# Autodesk Inventor assembly: keyboard-mockup_cherrymx
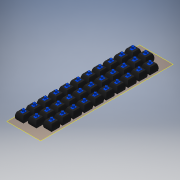
[picture p0: Inventor's stored thumbnail of the model, 180x180]
Saved by Autodesk Inventor 2016 (Build 200138000, 138)
## iProperties
Created: 2016-12-08
Part Number: keyboard-mockup_cherrymx
Document SubType Name: Assembly
Designer: Cemra JC
Author: Cemra JC
## Documents named in this file (2)
- J:\The Files\The Software Files\Projects\stenotoppers\cherrymx\base-model\keyboard-mockup_cherrymx.iam
- J:\The Files\The Software Files\Projects\stenotoppers\cherrymx\base-model\keyswitch_cherrymx.iam
## Components (32 placed, 1 different names)
1. keyswitch_cherrymx:3 [sub-assembly] — XZ-Constrain Row 1, Row 1 to Row 2 (vertical)
2. keyswitch_cherrymx:4 [sub-assembly]
3. keyswitch_cherrymx:5 [sub-assembly]
4. keyswitch_cherrymx:6 [sub-assembly]
5. keyswitch_cherrymx:7 [sub-assembly]
6. keyswitch_cherrymx:8 [sub-assembly]
7. keyswitch_cherrymx:9 [sub-assembly]
8. keyswitch_cherrymx:10 [sub-assembly]
9. keyswitch_cherrymx:11 [sub-assembly]
10. keyswitch_cherrymx:12 [sub-assembly]
11. keyswitch_cherrymx:13 [sub-assembly]
12. keyswitch_cherrymx:2 [sub-assembly] — XZ-Constrain Row 2, Row 1 to Row 2 (vertical), Row 2 to Row 3 (vertical)
13. keyswitch_cherrymx:14 [sub-assembly]
14. keyswitch_cherrymx:15 [sub-assembly]
15. keyswitch_cherrymx:16 [sub-assembly]
16. keyswitch_cherrymx:17 [sub-assembly]
17. keyswitch_cherrymx:18 [sub-assembly]
18. keyswitch_cherrymx:19 [sub-assembly]
19. keyswitch_cherrymx:20 [sub-assembly]
20. keyswitch_cherrymx:21 [sub-assembly]
21. keyswitch_cherrymx:22 [sub-assembly]
22. keyswitch_cherrymx:23 [sub-assembly]
23. keyswitch_cherrymx:1 [sub-assembly] — XZ-Constrain Row 3, Row 2 to Row 3 (vertical)
24. keyswitch_cherrymx:24 [sub-assembly]
25. keyswitch_cherrymx:25 [sub-assembly]
26. keyswitch_cherrymx:26 [sub-assembly]
27. keyswitch_cherrymx:27 [sub-assembly]
28. keyswitch_cherrymx:28 [sub-assembly]
29. keyswitch_cherrymx:29 [sub-assembly]
30. keyswitch_cherrymx:30 [sub-assembly]
31. keyswitch_cherrymx:31 [sub-assembly]
32. keyswitch_cherrymx:32 [sub-assembly]
## Component patterns: Row 1 (11 elements), Row 2 (11 elements), Row 3 (10 elements)
## Relationships (5: Mate 5)
- XZ-Constrain Row 1 [Mate]: keyswitch_cherrymx:3
- XZ-Constrain Row 2 [Mate]: keyswitch_cherrymx:2
- XZ-Constrain Row 3 [Mate]: keyswitch_cherrymx:1
- Row 1 to Row 2 (vertical) [Mate] (5 mm): keyswitch_cherrymx:3 ↔ keyswitch_cherrymx:2
- Row 2 to Row 3 (vertical) [Mate] (5 mm): keyswitch_cherrymx:2 ↔ keyswitch_cherrymx:1
